# Autodesk Inventor assembly: base-weel-2
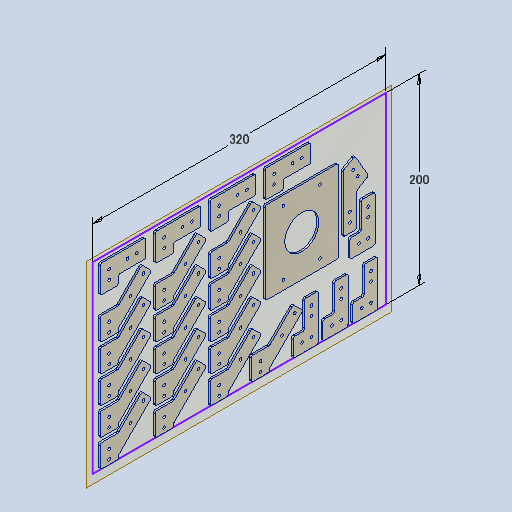
[picture p0: Inventor's stored thumbnail of the model, 512x512]
Saved by Autodesk Inventor 2025.2 (Build 292293000, 293)
## iProperties
Created: 2025-01-14
Part Number: base-weel-2
Document SubType Name: Assembly
Designer: haruy
Author: haruy
## Documents named in this file (6)
- C:\Users\haruy\Documents\ロボコン\NHK2025\cad\cnc\base-weel-2.iam
- C:\Users\haruy\Documents\ロボコン\NHK2025\cad\nagahisa\base_weel\base_weel-v2-Plate-3.ipt
- C:\Users\haruy\Documents\ロボコン\NHK2025\cad\nagahisa\base_weel\base_weel-v2-Plate-4.ipt
- C:\Users\haruy\Documents\ロボコン\NHK2025\cad\nagahisa\base_weel\base_weel-v2-Plate-1.ipt
- C:\Users\haruy\Documents\ロボコン\NHK2025\cad\nagahisa\base_weel\base_weel-v2-Plate-8.ipt
- C:\Users\haruy\Documents\ロボコン\NHK2025\cad\nagahisa\belt_liner\belt_liner_v2_Plate_20.ipt
## Components (26 placed, 5 different names)
1. base_weel-v2-Plate-3:17 — フラッシュ:4, フラッシュ:5, フラッシュ:6, フラッシュ:12
2. base_weel-v2-Plate-1:1 — フラッシュ:9, メイト:2, フラッシュ:10, メイト:7
3. base_weel-v2-Plate-8:4 — フラッシュ:13, メイト:8, メイト:9
4. belt_liner_v2_Plate_20:2 — フラッシュ:15, メイト:7, メイト:8, メイト:9
5. base_weel-v2-Plate-3:1 — フラッシュ:1, フラッシュ:3, メイト:1
6. base_weel-v2-Plate-3:7
7. base_weel-v2-Plate-3:12 — フラッシュ:5, フラッシュ:6
8. base_weel-v2-Plate-4:1 — フラッシュ:7, フラッシュ:8
9. base_weel-v2-Plate-4:2
10. base_weel-v2-Plate-4:3
11. base_weel-v2-Plate-4:4 — メイト:2, フラッシュ:10
12. base_weel-v2-Plate-8:1 — フラッシュ:11, フラッシュ:12
13. base_weel-v2-Plate-8:2
14. base_weel-v2-Plate-8:3
15. base_weel-v2-Plate-3:2 — フラッシュ:2, フラッシュ:3, メイト:1
16. base_weel-v2-Plate-3:4
17. base_weel-v2-Plate-3:5
18. base_weel-v2-Plate-3:6 — フラッシュ:8
19. base_weel-v2-Plate-3:8
20. base_weel-v2-Plate-3:9
21. base_weel-v2-Plate-3:10
22. base_weel-v2-Plate-3:11
23. base_weel-v2-Plate-3:13
24. base_weel-v2-Plate-3:14
25. base_weel-v2-Plate-3:15
26. base_weel-v2-Plate-3:16
## Component patterns: (3 elements, first: base_weel-v2-Plate-3:1), (4 elements, first: base_weel-v2-Plate-4:1), (3 elements, first: base_weel-v2-Plate-8:1), (4 elements, first: base_weel-v2-Plate-3:2), コンポーネント パターン 1:2 (4 elements), コンポーネント パターン 1:3 (4 elements)
## Relationships (19: Flush 14, Mate 5)
- フラッシュ:1 [Flush]: base_weel-v2-Plate-3:1
- フラッシュ:2 [Flush]: base_weel-v2-Plate-3:2
- フラッシュ:3 [Flush]: base_weel-v2-Plate-3:1 ↔ base_weel-v2-Plate-3:2
- メイト:1 [Mate] (5 mm): base_weel-v2-Plate-3:1 ↔ base_weel-v2-Plate-3:2
- フラッシュ:4 [Flush]: base_weel-v2-Plate-3:17
- フラッシュ:5 [Flush]: base_weel-v2-Plate-3:17 ↔ base_weel-v2-Plate-3:12
- フラッシュ:6 [Flush] (-45 mm): base_weel-v2-Plate-3:17 ↔ base_weel-v2-Plate-3:12
- フラッシュ:7 [Flush]: base_weel-v2-Plate-4:1
- フラッシュ:8 [Flush]: base_weel-v2-Plate-4:1 ↔ base_weel-v2-Plate-3:6
- フラッシュ:9 [Flush]: base_weel-v2-Plate-1:1
- メイト:2 [Mate] (5 mm): base_weel-v2-Plate-1:1 ↔ base_weel-v2-Plate-4:4
- フラッシュ:10 [Flush]: base_weel-v2-Plate-1:1 ↔ base_weel-v2-Plate-4:4
- フラッシュ:11 [Flush]: base_weel-v2-Plate-8:1
- フラッシュ:12 [Flush]: base_weel-v2-Plate-3:17 ↔ base_weel-v2-Plate-8:1
- フラッシュ:13 [Flush]: base_weel-v2-Plate-8:4
- フラッシュ:15 [Flush]: belt_liner_v2_Plate_20:2
- メイト:7 [Mate] (5 mm): base_weel-v2-Plate-1:1 ↔ belt_liner_v2_Plate_20:2
- メイト:8 [Mate] (5 mm): base_weel-v2-Plate-8:4 ↔ belt_liner_v2_Plate_20:2
- メイト:9 [Mate] (5 mm): base_weel-v2-Plate-8:4 ↔ belt_liner_v2_Plate_20:2
